# Autodesk Inventor assembly: main room, doors, corridor connected
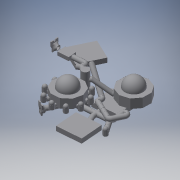
[picture p0: Inventor's stored thumbnail of the model, 180x180]
Saved by Autodesk Inventor 2017 (Build 210142000, 142)
## iProperties
Created: 2018-03-04
Part Number: main room, doors, corridor connected
Document SubType Name: Assembly
Designer: Braxton
Author: Braxton
## Documents named in this file (21)
- E:\School\Game develpment\geoscape\done\double wall\map (double wall)\main room, doors, corridor connected (two walls).iam
- E:\School\Game develpment\geoscape\done\single wall\rooms  (one wall)\assembly\main room with double door.iam
- E:\School\Game develpment\geoscape\done\double wall\corridors (double wall)\corridor (two walls).ipt
- E:\School\Game develpment\geoscape\done\double wall\corridors (double wall)\corridor turn (two walls).ipt
- E:\School\Game develpment\geoscape\done\double wall\corridors (double wall)\Y corridor (two walls).ipt
- E:\School\Game develpment\geoscape\done\double wall\corridors (double wall)\end cap (two walls).ipt
- E:\School\Game develpment\geoscape\done\double wall\corridors (double wall)\ramp top connect (two walls).ipt
- E:\School\Game develpment\geoscape\done\double wall\corridors (double wall)\ramp (two walls).ipt
- E:\School\Game develpment\geoscape\done\double wall\corridors (double wall)\ramp bottom connect (two walls).ipt
- E:\School\Game develpment\geoscape\done\double wall\corridors (double wall)\curve ramp (two walls).ipt
- E:\School\Game develpment\geoscape\done\single wall\rooms  (one wall)\assembly\dome with double door.iam
- E:\School\Game develpment\geoscape\done\double wall\corridors (double wall)\X corridor (two walls).ipt
- E:\School\Game develpment\geoscape\done\double wall\rooms (double wall)\room with 15 cubicals (two walls).ipt
- E:\School\Game develpment\geoscape\done\double wall\corridors (double wall)\ramp connect both ends (two walls).ipt
- E:\School\Game develpment\geoscape\done\doors\end door\9 foot door\end door room (9).ipt
- E:\School\Game develpment\geoscape\done\doors\end door\9 foot door\end door assembly (9).ipt.iam
- E:\School\Game develpment\geoscape\done\single wall\rooms  (one wall)\assembly\dome one terminal.iam
- E:\School\Game develpment\geoscape\done\single wall\rooms  (one wall)\assembly\assembly of dome with corridors with all doors.iam
- E:\School\Game develpment\geoscape\done\doors\end door\9 foot door\end door assembly (closed) (9).ipt.iam
- end door assembly (9).ipt
- end door assembly (closed) (9).ipt
## Components (69 placed, 19 different names)
1. room with 15 cubicals (two walls):3 — Flush:103, Insert:87
2. ramp top connect (two walls):3 — Flush:84, Insert:77, Flush:103, Insert:87
3. ramp (two walls):8 — Insert:74, Flush:81, Insert:75, Flush:82
4. ramp (two walls):7 — Insert:75, Flush:82, Insert:76, Flush:83
5. ramp (two walls):6 — Insert:73, Flush:80, Flush:84, Insert:77
6. ramp (two walls):5 — Insert:72, Flush:79, Insert:73, Flush:80
7. ramp (two walls):4 — Insert:72, Flush:79, Insert:74, Flush:81
8. ramp bottom connect (two walls):3 — Insert:71, Flush:78, Insert:76, Flush:83
9. corridor turn (two walls):8 — Insert:70, Flush:77, Insert:71, Flush:78
10. corridor turn (two walls):7 — Flush:75, Insert:68, Insert:70, Flush:77
11. corridor (two walls):18 — Flush:71, Insert:64, Flush:75, Insert:68
12. corridor (two walls):17 — Insert:65, Flush:72, Insert:66, Flush:73
13. corridor (two walls):16 — Insert:66, Flush:73, Flush:74, Insert:67
14. corridor (two walls):15 — Flush:71, Insert:64, Insert:65, Flush:72
15. corridor turn (two walls):6 — Flush:70, Insert:63, Flush:74, Insert:67
16. corridor (two walls):14 — Flush:68, Insert:61, Flush:70, Insert:63
17. corridor (two walls):13 — Flush:68, Insert:61, Insert:62, Flush:69
18. ramp top connect (two walls):2 — Flush:65, Insert:58, Flush:66, Insert:60
19. corridor turn (two walls):5 — Flush:67, Insert:59, Insert:62, Flush:69
20. corridor turn (two walls):4 — Flush:66, Flush:67, Insert:59, Insert:60
21. ramp bottom connect (two walls):2 — Flush:64, Insert:57, Flush:65, Insert:58
22. corridor (two walls):12 — Flush:56, Insert:50, Insert:51, Flush:60
23. corridor (two walls):11 — Insert:52, Insert:53, Flush:57, Flush:58
24. corridor (two walls):10 — Insert:53, Flush:57, Flush:59, Flush:61, Insert:55
25. room with 15 cubicals (two walls):2 — Flush:49, Insert:48
26. ramp connect both ends (two walls):2 — Flush:46, Insert:45, Flush:48, Insert:47
27. ramp connect both ends (two walls):1 — Flush:47, Insert:46, Flush:49, Insert:48
28. room with 15 cubicals (two walls):1 — Flush:48, Insert:47
29. Y corridor (two walls):2 — Insert:51, Insert:52, Flush:58, Flush:60, Flush:64, Insert:57
30. X corridor (two walls):1 — Flush:44, Insert:43, Flush:46, Flush:47, Insert:45, Insert:46, Flush:56, Insert:50
31. corridor (two walls):9 — Flush:43, Flush:44, Insert:42, Insert:43
32. corridor (two walls):8 — Flush:42, Flush:43, Insert:41, Insert:42
33. corridor turn (two walls):3 — Insert:40, Flush:41, Flush:42, Insert:41
34. curve ramp (two walls):1 — Flush:23, Insert:24, Flush:24, Insert:25, Flush:33, Insert:27, Flush:35, Insert:36, Flush:38, Insert:37, Insert:40, Flush:41, Flush:76, Insert:69
35. ramp top connect (two walls):1 — Flush:24, Insert:25, Flush:25, Insert:26
36. corridor turn (two walls):2 — Flush:28, Flush:33, Insert:27, Insert:28
37. corridor (two walls):3 — Flush:28, Flush:29, Insert:32, Flush:54, Insert:49
38. corridor (two walls):4 — Flush:29, Flush:30, Insert:31, Insert:32
39. corridor (two walls):5 — Flush:30, Flush:31, Insert:30, Insert:31
40. corridor (two walls):6 — Flush:31, Flush:32, Insert:29, Insert:30
41. corridor (two walls):7 — Flush:32, Insert:28, Insert:29
42. end cap (two walls):4 — Flush:35, Insert:36
43. end cap (two walls):5 — Flush:38, Insert:37
44. ramp bottom connect (two walls):1 — Flush:19, Insert:18, Flush:40, Insert:39
45. ramp (two walls):1 — Flush:17, Insert:20, Flush:25, Insert:26
46. ramp (two walls):2 — Flush:17, Flush:18, Insert:19, Insert:20
47. ramp (two walls):3 — Flush:18, Flush:19, Insert:18, Insert:19
48. corridor (two walls):1 — Flush:1, Flush:2, Insert:1, Insert:2
49. corridor (two walls):2 — Flush:2, Flush:3, Insert:2, Insert:3
50. corridor turn (two walls):1 — Flush:3, Flush:4, Insert:3, Insert:4
51. Y corridor (two walls):1 — Flush:4, Insert:4, Flush:23, Insert:24, Flush:104, Insert:88
52. end cap (two walls):1 — Flush:104, Insert:88
53. dome one terminal:10 [sub-assembly] — Insert:81, Flush:93
54. dome one terminal:9 [sub-assembly] — Insert:82, Flush:92
55. dome one terminal:8 [sub-assembly] — Insert:83, Flush:91
56. dome one terminal:7 [sub-assembly] — Insert:86, Flush:90
57. dome one terminal:6 [sub-assembly] — Insert:85, Flush:89
58. dome one terminal:5 [sub-assembly] — Insert:84, Flush:88
59. dome one terminal:4 [sub-assembly] — Insert:80, Flush:87
60. dome one terminal:3 [sub-assembly] — Insert:79, Flush:86
61. dome one terminal:2 [sub-assembly] — Insert:78, Flush:85
62. assembly of dome with corridors with all doors:1 [sub-assembly] — Flush:76, Insert:69, Insert:78, Insert:79, Insert:80, Insert:81, Insert:82, Insert:83, Insert:84, Insert:85, Insert:86, Flush:85, Flush:86, Flush:87, Flush:88, Flush:89, Flush:90, Flush:91, Flush:92, Flush:93
63. dome one terminal:1 [sub-assembly] — Flush:59, Flush:61, Insert:55
64. dome with double door:1 [sub-assembly] — Flush:40, Insert:39
65. main room with double door:1 [sub-assembly] — Flush:1, Insert:1, Flush:106, Insert:89
66. end door assembly (closed) (9).ipt:2 [sub-assembly] — Mate:55, Mate:56
67. end door room (9):1 — Flush:54, Insert:49, Flush:55, Mate:47, Mate:48, Mate:51, Mate:52
68. end door assembly (9).ipt:1 [sub-assembly] — Flush:55, Mate:47, Mate:48, Mate:51, Mate:52
69. end door room (Starting) (9):2 — Flush:106, Insert:89, Mate:55, Mate:56
## Relationships (140: Flush 68, Insert 66, Mate 6)
- Flush:1: corridor (two walls):1 ↔ main room with double door:1
- Flush:2: corridor (two walls):1 ↔ corridor (two walls):2
- Flush:3: corridor (two walls):2 ↔ corridor turn (two walls):1
- Flush:4: corridor turn (two walls):1 ↔ Y corridor (two walls):1
- Insert:1: corridor (two walls):1 ↔ main room with double door:1
- Insert:2: corridor (two walls):1 ↔ corridor (two walls):2
- Insert:3: corridor (two walls):2 ↔ corridor turn (two walls):1
- Insert:4: corridor turn (two walls):1 ↔ Y corridor (two walls):1
- Flush:17: ramp (two walls):1 ↔ ramp (two walls):2
- Flush:18: ramp (two walls):2 ↔ ramp (two walls):3
- Flush:19: ramp bottom connect (two walls):1 ↔ ramp (two walls):3
- Insert:18: ramp bottom connect (two walls):1 ↔ ramp (two walls):3
- Insert:19: ramp (two walls):2 ↔ ramp (two walls):3
- Insert:20: ramp (two walls):1 ↔ ramp (two walls):2
- Flush:23: curve ramp (two walls):1 ↔ Y corridor (two walls):1
- Insert:24: curve ramp (two walls):1 ↔ Y corridor (two walls):1
- Flush:24: curve ramp (two walls):1 ↔ ramp top connect (two walls):1
- Insert:25: curve ramp (two walls):1 ↔ ramp top connect (two walls):1
- Flush:25: ramp top connect (two walls):1 ↔ ramp (two walls):1
- Insert:26: ramp top connect (two walls):1 ↔ ramp (two walls):1
- Flush:28: corridor turn (two walls):2 ↔ corridor (two walls):3
- Flush:29: corridor (two walls):3 ↔ corridor (two walls):4
- Flush:30: corridor (two walls):4 ↔ corridor (two walls):5
- Flush:31: corridor (two walls):5 ↔ corridor (two walls):6
- Flush:32: corridor (two walls):6 ↔ corridor (two walls):7
- Flush:33: curve ramp (two walls):1 ↔ corridor turn (two walls):2
- Insert:27: curve ramp (two walls):1 ↔ corridor turn (two walls):2
- Insert:28: corridor turn (two walls):2 ↔ corridor (two walls):7
- Insert:29: corridor (two walls):6 ↔ corridor (two walls):7
- Insert:30: corridor (two walls):5 ↔ corridor (two walls):6
- Insert:31: corridor (two walls):4 ↔ corridor (two walls):5
- Insert:32: corridor (two walls):3 ↔ corridor (two walls):4
- Flush:35: curve ramp (two walls):1 ↔ end cap (two walls):4
- Insert:36: curve ramp (two walls):1 ↔ end cap (two walls):4
- Flush:38: curve ramp (two walls):1 ↔ end cap (two walls):5
- Insert:37: curve ramp (two walls):1 ↔ end cap (two walls):5
- Flush:40: ramp bottom connect (two walls):1 ↔ dome with double door:1
- Insert:39: ramp bottom connect (two walls):1 ↔ dome with double door:1
- Insert:40: corridor turn (two walls):3 ↔ curve ramp (two walls):1
- Flush:41: corridor turn (two walls):3 ↔ curve ramp (two walls):1
- Flush:42: corridor (two walls):8 ↔ corridor turn (two walls):3
- Flush:43: corridor (two walls):9 ↔ corridor (two walls):8
- Flush:44: X corridor (two walls):1 ↔ corridor (two walls):9
- Insert:41: corridor (two walls):8 ↔ corridor turn (two walls):3
- Insert:42: corridor (two walls):9 ↔ corridor (two walls):8
- Insert:43: X corridor (two walls):1 ↔ corridor (two walls):9
- Flush:46: ramp connect both ends (two walls):2 ↔ X corridor (two walls):1
- Flush:47: ramp connect both ends (two walls):1 ↔ X corridor (two walls):1
- Insert:45: ramp connect both ends (two walls):2 ↔ X corridor (two walls):1
- Insert:46: ramp connect both ends (two walls):1 ↔ X corridor (two walls):1
- Flush:48: ramp connect both ends (two walls):2 ↔ room with 15 cubicals (two walls):1
- Insert:47: ramp connect both ends (two walls):2 ↔ room with 15 cubicals (two walls):1
- Flush:49: room with 15 cubicals (two walls):2 ↔ ramp connect both ends (two walls):1
- Insert:48: room with 15 cubicals (two walls):2 ↔ ramp connect both ends (two walls):1
- Flush:54: corridor (two walls):3 ↔ end door room (9):1
- Insert:49: corridor (two walls):3 ↔ end door room (9):1
- Flush:55: end door room (9):1 ↔ end door assembly (9).ipt:1
- Mate:47: end door room (9):1 ↔ end door assembly (9).ipt:1
- Mate:48: end door room (9):1 ↔ end door assembly (9).ipt:1
- Flush:56: corridor (two walls):12 ↔ X corridor (two walls):1
- Insert:50: corridor (two walls):12 ↔ X corridor (two walls):1
- Insert:51: corridor (two walls):12 ↔ Y corridor (two walls):2
- Insert:52: corridor (two walls):11 ↔ Y corridor (two walls):2
- Insert:53: corridor (two walls):11 ↔ corridor (two walls):10
- Flush:57: corridor (two walls):11 ↔ corridor (two walls):10
- Flush:58: corridor (two walls):11 ↔ Y corridor (two walls):2
- Flush:59: corridor (two walls):10 ↔ dome one terminal:1
- Flush:60: corridor (two walls):12 ↔ Y corridor (two walls):2
- Flush:61: corridor (two walls):10 ↔ dome one terminal:1
- Insert:55: corridor (two walls):10 ↔ dome one terminal:1
- Flush:64: ramp bottom connect (two walls):2 ↔ Y corridor (two walls):2
- Insert:57: ramp bottom connect (two walls):2 ↔ Y corridor (two walls):2
- Flush:65: ramp top connect (two walls):2 ↔ ramp bottom connect (two walls):2
- Insert:58: ramp top connect (two walls):2 ↔ ramp bottom connect (two walls):2
- Flush:66: ramp top connect (two walls):2 ↔ corridor turn (two walls):4
- Flush:67: corridor turn (two walls):5 ↔ corridor turn (two walls):4
- Insert:59: corridor turn (two walls):5 ↔ corridor turn (two walls):4
- Insert:60: ramp top connect (two walls):2 ↔ corridor turn (two walls):4
- Flush:68: corridor (two walls):14 ↔ corridor (two walls):13
- Insert:61: corridor (two walls):14 ↔ corridor (two walls):13
- Insert:62: corridor (two walls):13 ↔ corridor turn (two walls):5
- Flush:69: corridor (two walls):13 ↔ corridor turn (two walls):5
- Flush:70: corridor turn (two walls):6 ↔ corridor (two walls):14
- Insert:63: corridor turn (two walls):6 ↔ corridor (two walls):14
- Flush:71: corridor (two walls):18 ↔ corridor (two walls):15
- Insert:64: corridor (two walls):18 ↔ corridor (two walls):15
- Insert:65: corridor (two walls):17 ↔ corridor (two walls):15
- Flush:72: corridor (two walls):17 ↔ corridor (two walls):15
- Insert:66: corridor (two walls):17 ↔ corridor (two walls):16
- Flush:73: corridor (two walls):17 ↔ corridor (two walls):16
- Flush:74: corridor (two walls):16 ↔ corridor turn (two walls):6
- Insert:67: corridor (two walls):16 ↔ corridor turn (two walls):6
- Mate:51: end door room (9):1 ↔ end door assembly (9).ipt:1
- Mate:52: end door room (9):1 ↔ end door assembly (9).ipt:1
- Flush:75: corridor turn (two walls):7 ↔ corridor (two walls):18
- Insert:68: corridor turn (two walls):7 ↔ corridor (two walls):18
- Flush:76: curve ramp (two walls):1 ↔ assembly of dome with corridors with all doors:1
- Insert:69: curve ramp (two walls):1 ↔ assembly of dome with corridors with all doors:1
- Insert:70: corridor turn (two walls):8 ↔ corridor turn (two walls):7
- Flush:77: corridor turn (two walls):8 ↔ corridor turn (two walls):7
- Insert:71: ramp bottom connect (two walls):3 ↔ corridor turn (two walls):8
- Flush:78: ramp bottom connect (two walls):3 ↔ corridor turn (two walls):8
- Insert:72: ramp (two walls):5 ↔ ramp (two walls):4
- Flush:79: ramp (two walls):5 ↔ ramp (two walls):4
- Insert:73: ramp (two walls):6 ↔ ramp (two walls):5
- Flush:80: ramp (two walls):6 ↔ ramp (two walls):5
- Insert:74: ramp (two walls):8 ↔ ramp (two walls):4
- Flush:81: ramp (two walls):8 ↔ ramp (two walls):4
- Insert:75: ramp (two walls):8 ↔ ramp (two walls):7
- Flush:82: ramp (two walls):8 ↔ ramp (two walls):7
- Insert:76: ramp (two walls):7 ↔ ramp bottom connect (two walls):3
- Flush:83: ramp (two walls):7 ↔ ramp bottom connect (two walls):3
- Flush:84: ramp top connect (two walls):3 ↔ ramp (two walls):6
- Insert:77: ramp top connect (two walls):3 ↔ ramp (two walls):6
- Insert:78: dome one terminal:2 ↔ assembly of dome with corridors with all doors:1
- Insert:79: dome one terminal:3 ↔ assembly of dome with corridors with all doors:1
- Insert:80: dome one terminal:4 ↔ assembly of dome with corridors with all doors:1
- Insert:81: dome one terminal:10 ↔ assembly of dome with corridors with all doors:1
- Insert:82: dome one terminal:9 ↔ assembly of dome with corridors with all doors:1
- Insert:83: dome one terminal:8 ↔ assembly of dome with corridors with all doors:1
- Insert:84: dome one terminal:5 ↔ assembly of dome with corridors with all doors:1
- Insert:85: dome one terminal:6 ↔ assembly of dome with corridors with all doors:1
- Insert:86: dome one terminal:7 ↔ assembly of dome with corridors with all doors:1
- Flush:85: dome one terminal:2 ↔ assembly of dome with corridors with all doors:1
- Flush:86: dome one terminal:3 ↔ assembly of dome with corridors with all doors:1
- Flush:87: dome one terminal:4 ↔ assembly of dome with corridors with all doors:1
- Flush:88: dome one terminal:5 ↔ assembly of dome with corridors with all doors:1
- Flush:89: dome one terminal:6 ↔ assembly of dome with corridors with all doors:1
- Flush:90: dome one terminal:7 ↔ assembly of dome with corridors with all doors:1
- Flush:91: dome one terminal:8 ↔ assembly of dome with corridors with all doors:1
- Flush:92: dome one terminal:9 ↔ assembly of dome with corridors with all doors:1
- Flush:93: dome one terminal:10 ↔ assembly of dome with corridors with all doors:1
- Flush:103: room with 15 cubicals (two walls):3 ↔ ramp top connect (two walls):3
- Insert:87: room with 15 cubicals (two walls):3 ↔ ramp top connect (two walls):3
- Flush:104: Y corridor (two walls):1 ↔ end cap (two walls):1
- Insert:88: Y corridor (two walls):1 ↔ end cap (two walls):1
- Flush:106: main room with double door:1 ↔ end door room (Starting) (9):2
- Insert:89: main room with double door:1 ↔ end door room (Starting) (9):2
- Mate:55: end door assembly (closed) (9).ipt:2 ↔ end door room (Starting) (9):2
- Mate:56: end door assembly (closed) (9).ipt:2 ↔ end door room (Starting) (9):2
